# Autodesk Inventor assembly: Snow Blower Tire with Gear Box and Mini-CIM
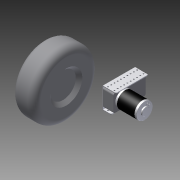
[picture p0: Inventor's stored thumbnail of the model, 180x180]
Saved by Autodesk Inventor 2015 (Build 190159000, 159)
## iProperties
Created: 2016-01-21
Part Number: Snow Blower Tire with Gear Box and Mini-CIM
Document SubType Name: Assembly
Designer: sethbattis
Author: sethbattis
## Documents named in this file (6)
- \\area51\team3566\cad\FRC 2016\Snow Blower Tire with Gear Box and Mini-CIM.iam
- \\area51\team3566\cad\FRC 2016\Imported Components\MOT_MiniCIMMotor_217-3371.ipt\MOT_MiniCIMMotor_217-3371.ipt.ipt
- \\area51\team3566\cad\FRC 2016\Snow Blower Tire.ipt
- \\area51\team3566\cad\FRC 2016\am-2679 671 Mecanum Gearbox.ipt
- \\area51\team3566\cad\FRC 2016\AM14U3 End Sheet 5in.ipt
- MOT_MiniCIMMotor_217-3371.ipt
## Components (4 placed, 4 different names)
1. MOT_MiniCIMMotor_217-3371.ipt:1 — Mate:1, Mate:2
2. Snow Blower Tire:1
3. am-2679 671 Mecanum Gearbox:1 — Mate:1, Mate:2, Mate:3, Flush:1
4. AM14U3 End Sheet 5in:1 — Mate:3, Flush:1
## Relationships (4: Mate 3, Flush 1)
- Mate:1: MOT_MiniCIMMotor_217-3371.ipt:1 ↔ am-2679 671 Mecanum Gearbox:1
- Mate:2: MOT_MiniCIMMotor_217-3371.ipt:1 ↔ am-2679 671 Mecanum Gearbox:1
- Mate:3: am-2679 671 Mecanum Gearbox:1 ↔ AM14U3 End Sheet 5in:1
- Flush:1: am-2679 671 Mecanum Gearbox:1 ↔ AM14U3 End Sheet 5in:1
